# Autodesk Inventor assembly: volume_under
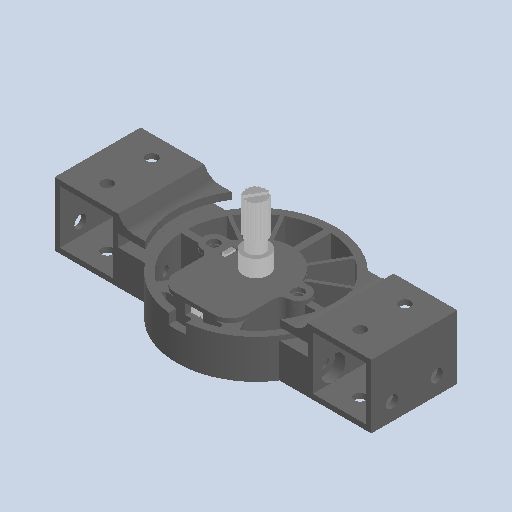
[picture p0: Inventor's stored thumbnail of the model, 512x512]
Saved by Autodesk Inventor 2026.1 (Build 301233020, 233B)
## iProperties
Created: 2026-02-02
Part Number: volume_under
Document SubType Name: Assembly
Designer: hibik
Author: hibik
## Documents named in this file (5)
- C:\Users\hibik\Documents\Robomech\HR\controller\hard\body\volume_under.iam
- C:\Users\hibik\Documents\Robomech\HR\controller\hard\body\volume_case_under.ipt
- C:\Users\hibik\Documents\Robomech\HR\controller\hard\body\volume.ipt
- C:\Users\hibik\Documents\Robomech\HR\controller\hard\body\volume_case_upper.ipt
- C:\Users\hibik\Documents\Robomech\HR\controller\hard\body\pole_setter_crow.ipt
## Components (5 placed, 4 different names)
1. volume_case_under:1 — 挿入:1, 角度:1, 挿入:2, 角度:2, 挿入:3, 挿入:4, 角度:3, 角度:4
2. volume:1 — 挿入:1, 角度:1
3. volume_case_upper:1 — 挿入:2, 角度:2
4. pole_setter_crow:1 — 挿入:3, 角度:4
5. pole_setter_crow:2 — 挿入:4, 角度:3
## Relationships (8: Insert 4, Angle 4)
- 挿入:1 [Insert]: volume_case_under:1 ↔ volume:1
- 角度:1 [Angle] (0 deg): volume_case_under:1 ↔ volume:1
- 挿入:2 [Insert]: volume_case_under:1 ↔ volume_case_upper:1
- 角度:2 [Angle] (0 deg): volume_case_under:1 ↔ volume_case_upper:1
- 挿入:3 [Insert]: volume_case_under:1 ↔ pole_setter_crow:1
- 挿入:4 [Insert]: volume_case_under:1 ↔ pole_setter_crow:2
- 角度:3 [Angle] (0 deg): volume_case_under:1 ↔ pole_setter_crow:2
- 角度:4 [Angle] (0 deg): volume_case_under:1 ↔ pole_setter_crow:1
